# Autodesk Inventor assembly: shaftSealAssembly
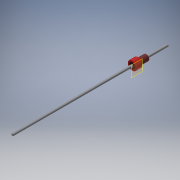
[picture p0: Inventor's stored thumbnail of the model, 180x180]
Saved by Autodesk Inventor 2018 (Build 220112000, 112)
## iProperties
Created: 2020-02-25
Part Number: shaftSealAssembly
Document SubType Name: Assembly
Designer: anirudh
Author: anirudh
## Documents named in this file (6)
- D:\Silicon Sharks\2019-2020\servoBox\shaftSeal\shaftSealAssembly.iam
- D:\Silicon Sharks\2019-2020\servoBox\shaftSeal\shaftSealBulkhead.ipt
- D:\Silicon Sharks\2019-2020\servoBox\shaftSeal\cupORing.ipt
- D:\Silicon Sharks\2019-2020\servoBox\shaftSeal\6362K111_WATER-RESISTANT DRY-RUNNING SLEEVE BEARING.ipt
- D:\Silicon Sharks\2019-2020\servoBox\shaftSeal\6362K211_WATER-RESISTANT DRY-RUNNING SLEEVE BEARING.ipt
- D:\Silicon Sharks\2019-2020\servoBox\shaftSeal\1257K530_MINIATURE 303 STAINLESS STEEL DRIVE SHAFT.ipt
## Components (7 placed, 5 different names)
1. shaftSealBulkhead:1 — Mate:9, Mate:10, Mate:11, Mate:12
2. cupORing:1 — Mate:1, Mate:2, Mate:3, Mate:4
3. cupORing:2 — Mate:5, Mate:6, Mate:7
4. 6362K111_WATER-RESISTANT DRY-RUNNING SLEEVE BEARING:1 — Mate:3, Mate:4, Mate:5, Mate:6, Mate:8
5. 6362K111_WATER-RESISTANT DRY-RUNNING SLEEVE BEARING:2 — Mate:7, Mate:8
6. 6362K211_WATER-RESISTANT DRY-RUNNING SLEEVE BEARING:1 — Mate:1, Mate:2, Mate:9, Mate:10
7. 1257K530_MINIATURE 303 STAINLESS STEEL DRIVE SHAFT:1 — Mate:11, Mate:12
## Relationships (12: Mate 12)
- Mate:1: cupORing:1 ↔ 6362K211_WATER-RESISTANT DRY-RUNNING SLEEVE BEARING:1
- Mate:2: cupORing:1 ↔ 6362K211_WATER-RESISTANT DRY-RUNNING SLEEVE BEARING:1
- Mate:3: cupORing:1 ↔ 6362K111_WATER-RESISTANT DRY-RUNNING SLEEVE BEARING:1
- Mate:4: cupORing:1 ↔ 6362K111_WATER-RESISTANT DRY-RUNNING SLEEVE BEARING:1
- Mate:5: cupORing:2 ↔ 6362K111_WATER-RESISTANT DRY-RUNNING SLEEVE BEARING:1
- Mate:6: cupORing:2 ↔ 6362K111_WATER-RESISTANT DRY-RUNNING SLEEVE BEARING:1
- Mate:7: cupORing:2 ↔ 6362K111_WATER-RESISTANT DRY-RUNNING SLEEVE BEARING:2
- Mate:8: 6362K111_WATER-RESISTANT DRY-RUNNING SLEEVE BEARING:1 ↔ 6362K111_WATER-RESISTANT DRY-RUNNING SLEEVE BEARING:2
- Mate:9: shaftSealBulkhead:1 ↔ 6362K211_WATER-RESISTANT DRY-RUNNING SLEEVE BEARING:1
- Mate:10: shaftSealBulkhead:1 ↔ 6362K211_WATER-RESISTANT DRY-RUNNING SLEEVE BEARING:1
- Mate:11: shaftSealBulkhead:1 ↔ 1257K530_MINIATURE 303 STAINLESS STEEL DRIVE SHAFT:1
- Mate:12 (-69.85 mm): shaftSealBulkhead:1 ↔ 1257K530_MINIATURE 303 STAINLESS STEEL DRIVE SHAFT:1
